# Autodesk Inventor assembly: Assembly1
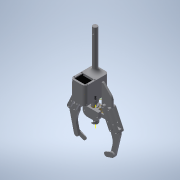
[picture p0: Inventor's stored thumbnail of the model, 180x180]
Saved by Autodesk Inventor 2020.1 (Build 241239000, 239)
## iProperties
Created: 2018-05-21
Part Number: Assembly1
Document SubType Name: Assembly
Designer: Bardo91
Author: Bardo91
## Documents named in this file (9)
- D:\programming\hecatonquiros\cad_models\tools\gripper\serial_model_0dof\Assembly1.iam
- D:\programming\hecatonquiros\cad_models\tools\gripper\serial_model_0dof\core_attachment.ipt
- D:\programming\hecatonquiros\cad_models\tools\gripper\serial_model_0dof\case_core.ipt
- D:\programming\hecatonquiros\cad_models\tools\gripper\serial_model_0dof\bar.ipt
- D:\programming\hecatonquiros\cad_models\tools\gripper\serial_model_0dof\gripper.ipt
- D:\programming\hecatonquiros\cad_models\tools\gripper\serial_model_0dof\ScrewActuatorGripper.ipt
- D:\programming\hecatonquiros\cad_models\tools\gripper\serial_model_0dof\ScrewActuatorGripperCenter.ipt
- D:\programming\hecatonquiros\cad_models\tools\gripper\serial_model_0dof\barMini.ipt
- D:\programming\hecatonquiros\cad_models\tools\gripper\serial_model_0dof\feetech_sc215.ipt
## Components (17 placed, 8 different names)
1. core_attachment:1 — Mate:1, Mate:2, Mate:3, Mate:10, Mate:11, Mate:17, Mate:18, Mate:24, Mate:25, Mate:39, Mate:40, Mate:41, Mate:42, Mate:49, Mate:50, Mate:51, Mate:60, Mate:61, Mate:62, Mate:63
2. case_core:1 — Mate:1, Mate:2, Mate:3
3. bar:2 — Mate:11, Mate:37, Mate:39, Mate:44
4. bar:4 — Mate:10, Mate:40, Mate:43, Mate:45
5. gripper:1 — Mate:43, Mate:44, Mate:52, Mate:53, Mate:58, Mate:59
6. ScrewActuatorGripper:1 — Mate:17, Mate:18, Mate:19
7. ScrewActuatorGripperCenter:1 — Mate:19, Mate:33, Mate:35
8. barMini:1 — Mate:35, Mate:37, Mate:45
9. barMini:2 — Mate:33, Mate:38, Mate:48
10. bar:5 — Mate:25, Mate:38, Mate:41, Mate:46, Mate:48
11. bar:6 — Mate:24, Mate:42, Mate:47
12. gripper:2 — Mate:46, Mate:47, Mate:54, Mate:55, Mate:56, Mate:57
13. feetech_sc215:1 — Mate:49, Mate:50, Mate:51
14. bar:7 — Mate:55, Mate:56, Mate:63
15. bar:8 — Mate:54, Mate:57, Mate:62
16. bar:9 — Mate:53, Mate:59, Mate:61
17. bar:10 — Mate:52, Mate:58, Mate:60
## Relationships (39: Mate 39)
- Mate:1: core_attachment:1 ↔ case_core:1
- Mate:2: core_attachment:1 ↔ case_core:1
- Mate:3: core_attachment:1 ↔ case_core:1
- Mate:10: core_attachment:1 ↔ bar:4
- Mate:11: core_attachment:1 ↔ bar:2
- Mate:17: core_attachment:1 ↔ ScrewActuatorGripper:1
- Mate:18: core_attachment:1 ↔ ScrewActuatorGripper:1
- Mate:19: ScrewActuatorGripper:1 ↔ ScrewActuatorGripperCenter:1
- Mate:24: core_attachment:1 ↔ bar:6
- Mate:25: core_attachment:1 ↔ bar:5
- Mate:33: ScrewActuatorGripperCenter:1 ↔ barMini:2
- Mate:35: ScrewActuatorGripperCenter:1 ↔ barMini:1
- Mate:37: bar:2 ↔ barMini:1
- Mate:38: barMini:2 ↔ bar:5
- Mate:39: core_attachment:1 ↔ bar:2
- Mate:40: core_attachment:1 ↔ bar:4
- Mate:41: core_attachment:1 ↔ bar:5
- Mate:42: core_attachment:1 ↔ bar:6
- Mate:43: bar:4 ↔ gripper:1
- Mate:44: bar:2 ↔ gripper:1
- Mate:45: bar:4 ↔ barMini:1
- Mate:46: bar:5 ↔ gripper:2
- Mate:47: bar:6 ↔ gripper:2
- Mate:48: barMini:2 ↔ bar:5
- Mate:49: core_attachment:1 ↔ feetech_sc215:1
- Mate:50: core_attachment:1 ↔ feetech_sc215:1
- Mate:51: core_attachment:1 ↔ feetech_sc215:1
- Mate:52: gripper:1 ↔ bar:10
- Mate:53: gripper:1 ↔ bar:9
- Mate:54: gripper:2 ↔ bar:8
- Mate:55: gripper:2 ↔ bar:7
- Mate:56: gripper:2 ↔ bar:7
- Mate:57: gripper:2 ↔ bar:8
- Mate:58: gripper:1 ↔ bar:10
- Mate:59: gripper:1 ↔ bar:9
- Mate:60: core_attachment:1 ↔ bar:10
- Mate:61: core_attachment:1 ↔ bar:9
- Mate:62: core_attachment:1 ↔ bar:8
- Mate:63: core_attachment:1 ↔ bar:7
